# Autodesk Inventor assembly: 中履组合
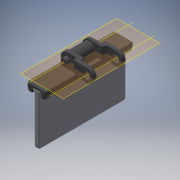
[picture p0: Inventor's stored thumbnail of the model, 180x180]
Saved by Autodesk Inventor 2019.4 (Build 234330000, 330)
## iProperties
Created: 2019-05-18
Part Number: 中履组合
Material: 常规
Document SubType Name: Assembly
Designer: aresp
Author: aresp
## Documents named in this file (3)
- C:\towerTakeOverCad\ncrCadLib\链轮履带\中履组合.iam
- C:\towerTakeOverCad\ncrCadLib\链轮履带\Chain Paddle Base.ipt
- C:\towerTakeOverCad\ncrCadLib\链轮履带\Chain Medium Paddle.ipt
## Components (2 placed, 2 different names)
1. Chain Medium Paddle:1 — 配合:1, 表面齐平:1, 配合:2
2. Chain Paddle Base:1 — 配合:1, 表面齐平:1, 配合:2
## Relationships (3: Mate 2, Flush 1)
- 配合:1 [Mate]: Chain Medium Paddle:1 ↔ Chain Paddle Base:1
- 表面齐平:1 [Flush]: Chain Medium Paddle:1 ↔ Chain Paddle Base:1
- 配合:2 [Mate] (0.1 mm): Chain Medium Paddle:1 ↔ Chain Paddle Base:1
